# Autodesk Inventor assembly: Robot
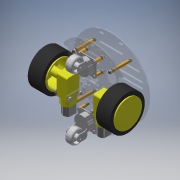
[picture p0: Inventor's stored thumbnail of the model, 180x180]
Saved by Autodesk Inventor 2018 (Build 220112000, 112)
## iProperties
Created: 2018-01-12
Part Number: Robot
Document SubType Name: Assembly
Designer: Kyle
Author: Kyle
## Documents named in this file (12)
- B:\My Documents\Project documentation\Hackathon-2018\Inventor\Robot\Robot.iam
- B:\My Documents\Project documentation\Hackathon-2018\Inventor\Robot\BottomPlate.ipt
- B:\My Documents\Project documentation\Hackathon-2018\Inventor\Robot\MotorMount.ipt
- B:\My Documents\Project documentation\Hackathon-2018\Inventor\Robot\MotorAssembly.iam
- B:\My Documents\Project documentation\Hackathon-2018\Inventor\Robot\MotorScrew.ipt
- B:\My Documents\Project documentation\Hackathon-2018\Inventor\Robot\Nut.ipt
- B:\My Documents\Project documentation\Hackathon-2018\Inventor\Robot\StandoffShort.ipt
- B:\My Documents\Project documentation\Hackathon-2018\Inventor\Robot\Castor.iam
- B:\My Documents\Project documentation\Hackathon-2018\Inventor\Robot\Screw.ipt
- B:\My Documents\Project documentation\Hackathon-2018\Inventor\Robot\StandoffLong.ipt
- B:\My Documents\Project documentation\Hackathon-2018\Inventor\Robot\TopPlate.ipt
- B:\My Documents\Project documentation\Hackathon-2018\Inventor\Robot\WheelAssembly.iam
## Components (52 placed, 11 different names)
1. BottomPlate:1 — Mate:1, Mate:2, Mate:3, Mate:4, Mate:5, Mate:6, Mate:7, Mate:8, Mate:9, Mate:10, Mate:11, Mate:12, Angle:1, Angle:2, Mate:33, Mate:34, Mate:35, Mate:36, Mate:37, Mate:38, Mate:39, Mate:40, Mate:41, Mate:43, Mate:45, Mate:47, Mate:60, Mate:61, Mate:62, Mate:63, Mate:64, Mate:65, Mate:66, Mate:67, Mate:79, Mate:80, Mate:81, Mate:82, Mate:83, Mate:84, Mate:85, Mate:86, Mate:87, Mate:89, Mate:91, Mate:93
2. MotorMount:1 — Mate:1, Mate:2, Mate:3, Mate:14, Mate:29, Mate:31
3. MotorMount:2 — Mate:4, Mate:5, Mate:6, Mate:13, Mate:21, Mate:23
4. MotorMount:3 — Mate:10, Mate:11, Mate:12, Mate:15, Mate:17, Mate:19
5. MotorMount:4 — Mate:7, Mate:8, Mate:9, Mate:16, Mate:25, Mate:27
6. MotorAssembly:1 [sub-assembly] — Mate:13, Angle:1, Mate:14, Mate:22, Mate:24, Mate:109, Mate:110, Mate:111
7. MotorAssembly:2 [sub-assembly] — Mate:15, Angle:2, Mate:16, Mate:18, Mate:20, Mate:106, Mate:107, Mate:108
8. MotorScrew:1 — Mate:17, Mate:18, Mate:26
9. MotorScrew:2 — Mate:19, Mate:20, Mate:28
10. MotorScrew:3 — Mate:23, Mate:24, Mate:30
11. MotorScrew:4 — Mate:21, Mate:22, Mate:32
12. Nut:1 — Mate:29, Mate:30
13. Nut:2 — Mate:31, Mate:32
14. Nut:3 — Mate:27, Mate:28
15. Nut:4 — Mate:25, Mate:26
16. StandoffShort:1 — Mate:36, Mate:40, Mate:42
17. StandoffShort:2 — Mate:35, Mate:37, Mate:48, Mate:50, Mate:51
18. StandoffShort:3 — Mate:34, Mate:39, Mate:44
19. StandoffShort:4 — Mate:33, Mate:38, Mate:46, Mate:49
20. Nut:5 — Mate:47, Mate:48
21. Nut:6 — Mate:45, Mate:46
22. Nut:7 — Mate:41, Mate:42
23. Nut:8 — Mate:43, Mate:44
24. Castor:1 [sub-assembly] — Mate:49, Mate:50, Mate:51, Mate:52, Mate:53, Mate:54, Mate:55, Mate:56, Mate:57, Mate:58, Mate:59
25. Screw:1 — Mate:52, Mate:54
26. Screw:2 — Mate:53, Mate:55
27. Screw:3 — Mate:56, Mate:59
28. Screw:4 — Mate:57, Mate:58
29. Castor:2 [sub-assembly] — Mate:68, Mate:69, Mate:70, Mate:71, Mate:72, Mate:73, Mate:74, Mate:76, Mate:77, Mate:78
30. StandoffShort:5 — Mate:60, Mate:65
31. StandoffShort:6 — Mate:61, Mate:67, Mate:68
32. StandoffShort:7 — Mate:62, Mate:66, Mate:69, Mate:70
33. StandoffShort:8 — Mate:63, Mate:64, Mate:75
34. Screw:5 — Mate:74, Mate:75
35. Screw:6 — Mate:73, Mate:76
36. Screw:7 — Mate:72, Mate:78
37. Screw:8 — Mate:71, Mate:77
38. StandoffLong:1 — Mate:79, Mate:82, Mate:88, Mate:95, Mate:96
39. StandoffLong:2 — Mate:80, Mate:81, Mate:90, Mate:97
40. StandoffLong:3 — Mate:83, Mate:84, Mate:94
41. StandoffLong:4 — Mate:85, Mate:86, Mate:92
42. Nut:9 — Mate:91, Mate:92
43. Nut:10 — Mate:93, Mate:94
44. Nut:11 — Mate:89, Mate:90
45. Nut:12 — Mate:87, Mate:88
46. TopPlate:1 — Mate:95, Mate:96, Mate:97, Mate:98, Mate:99, Mate:100, Mate:101, Mate:102, Mate:103, Mate:104, Mate:105
47. Screw:9 — Mate:98, Mate:99
48. Screw:10 — Mate:102, Mate:103
49. Screw:11 — Mate:100, Mate:101
50. Screw:12 — Mate:104, Mate:105
51. WheelAssembly:1 [sub-assembly] — Mate:106, Mate:107, Mate:108
52. WheelAssembly:2 [sub-assembly] — Mate:109, Mate:110, Mate:111
## Relationships (113: Mate 111, Angle 2)
- Mate:1: BottomPlate:1 ↔ MotorMount:1
- Mate:2: BottomPlate:1 ↔ MotorMount:1
- Mate:3: BottomPlate:1 ↔ MotorMount:1
- Mate:4: BottomPlate:1 ↔ MotorMount:2
- Mate:5: BottomPlate:1 ↔ MotorMount:2
- Mate:6: BottomPlate:1 ↔ MotorMount:2
- Mate:7: BottomPlate:1 ↔ MotorMount:4
- Mate:8: BottomPlate:1 ↔ MotorMount:4
- Mate:9: BottomPlate:1 ↔ MotorMount:4
- Mate:10: BottomPlate:1 ↔ MotorMount:3
- Mate:11: BottomPlate:1 ↔ MotorMount:3
- Mate:12: BottomPlate:1 ↔ MotorMount:3
- Mate:13: MotorMount:2 ↔ MotorAssembly:1
- Angle:1 (0 deg): BottomPlate:1 ↔ MotorAssembly:1
- Mate:14: MotorMount:1 ↔ MotorAssembly:1
- Mate:15: MotorMount:3 ↔ MotorAssembly:2
- Angle:2 (0 deg): BottomPlate:1 ↔ MotorAssembly:2
- Mate:16: MotorMount:4 ↔ MotorAssembly:2
- Mate:17: MotorMount:3 ↔ MotorScrew:1
- Mate:18: MotorAssembly:2 ↔ MotorScrew:1
- Mate:19: MotorMount:3 ↔ MotorScrew:2
- Mate:20: MotorAssembly:2 ↔ MotorScrew:2
- Mate:21: MotorMount:2 ↔ MotorScrew:4
- Mate:22: MotorAssembly:1 ↔ MotorScrew:4
- Mate:23: MotorMount:2 ↔ MotorScrew:3
- Mate:24: MotorAssembly:1 ↔ MotorScrew:3
- Mate:25: MotorMount:4 ↔ Nut:4
- Mate:26: MotorScrew:1 ↔ Nut:4
- Mate:27: MotorMount:4 ↔ Nut:3
- Mate:28: MotorScrew:2 ↔ Nut:3
- Mate:29: MotorMount:1 ↔ Nut:1
- Mate:30: MotorScrew:3 ↔ Nut:1
- Mate:31: MotorMount:1 ↔ Nut:2
- Mate:32: MotorScrew:4 ↔ Nut:2
- Mate:33: BottomPlate:1 ↔ StandoffShort:4
- Mate:34: BottomPlate:1 ↔ StandoffShort:3
- Mate:35: BottomPlate:1 ↔ StandoffShort:2
- Mate:36: BottomPlate:1 ↔ StandoffShort:1
- Mate:37: BottomPlate:1 ↔ StandoffShort:2
- Mate:38: BottomPlate:1 ↔ StandoffShort:4
- Mate:39: BottomPlate:1 ↔ StandoffShort:3
- Mate:40: BottomPlate:1 ↔ StandoffShort:1
- Mate:41: BottomPlate:1 ↔ Nut:7
- Mate:42: StandoffShort:1 ↔ Nut:7
- Mate:43: BottomPlate:1 ↔ Nut:8
- Mate:44: StandoffShort:3 ↔ Nut:8
- Mate:45: BottomPlate:1 ↔ Nut:6
- Mate:46: StandoffShort:4 ↔ Nut:6
- Mate:47: BottomPlate:1 ↔ Nut:5
- Mate:48: StandoffShort:2 ↔ Nut:5
- Mate:49: StandoffShort:4 ↔ Castor:1
- Mate:50: StandoffShort:2 ↔ Castor:1
- Mate:51: StandoffShort:2 ↔ Castor:1
- Mate:52: Castor:1 ↔ Screw:1
- Mate:53: Castor:1 ↔ Screw:2
- Mate:54: Castor:1 ↔ Screw:1
- Mate:55: Castor:1 ↔ Screw:2
- Mate:56: Castor:1 ↔ Screw:3
- Mate:57: Castor:1 ↔ Screw:4
- Mate:58: Castor:1 ↔ Screw:4
- Mate:59: Castor:1 ↔ Screw:3
- Mate:60: BottomPlate:1 ↔ StandoffShort:5
- Mate:61: BottomPlate:1 ↔ StandoffShort:6
- Mate:62: BottomPlate:1 ↔ StandoffShort:7
- Mate:63: BottomPlate:1 ↔ StandoffShort:8
- Mate:64: BottomPlate:1 ↔ StandoffShort:8
- Mate:65: BottomPlate:1 ↔ StandoffShort:5
- Mate:66: BottomPlate:1 ↔ StandoffShort:7
- Mate:67: BottomPlate:1 ↔ StandoffShort:6
- Mate:68: Castor:2 ↔ StandoffShort:6
- Mate:69: Castor:2 ↔ StandoffShort:7
- Mate:70: Castor:2 ↔ StandoffShort:7
- Mate:71: Castor:2 ↔ Screw:8
- Mate:72: Castor:2 ↔ Screw:7
- Mate:73: Castor:2 ↔ Screw:6
- Mate:74: Castor:2 ↔ Screw:5
- Mate:75: StandoffShort:8 ↔ Screw:5
- Mate:76: Castor:2 ↔ Screw:6
- Mate:77: Castor:2 ↔ Screw:8
- Mate:78: Castor:2 ↔ Screw:7
- Mate:79: BottomPlate:1 ↔ StandoffLong:1
- Mate:80: BottomPlate:1 ↔ StandoffLong:2
- Mate:81: BottomPlate:1 ↔ StandoffLong:2
- Mate:82: BottomPlate:1 ↔ StandoffLong:1
- Mate:83: BottomPlate:1 ↔ StandoffLong:3
- Mate:84: BottomPlate:1 ↔ StandoffLong:3
- Mate:85: BottomPlate:1 ↔ StandoffLong:4
- Mate:86: BottomPlate:1 ↔ StandoffLong:4
- Mate:87: BottomPlate:1 ↔ Nut:12
- Mate:88: StandoffLong:1 ↔ Nut:12
- Mate:89: BottomPlate:1 ↔ Nut:11
- Mate:90: StandoffLong:2 ↔ Nut:11
- Mate:91: BottomPlate:1 ↔ Nut:9
- Mate:92: StandoffLong:4 ↔ Nut:9
- Mate:93: BottomPlate:1 ↔ Nut:10
- Mate:94: StandoffLong:3 ↔ Nut:10
- Mate:95: StandoffLong:1 ↔ TopPlate:1
- Mate:96: StandoffLong:1 ↔ TopPlate:1
- Mate:97: StandoffLong:2 ↔ TopPlate:1
- Mate:98: TopPlate:1 ↔ Screw:9
- Mate:99: TopPlate:1 ↔ Screw:9
- Mate:100: TopPlate:1 ↔ Screw:11
- Mate:101: TopPlate:1 ↔ Screw:11
- Mate:102: TopPlate:1 ↔ Screw:10
- Mate:103: TopPlate:1 ↔ Screw:10
- Mate:104: TopPlate:1 ↔ Screw:12
- Mate:105: TopPlate:1 ↔ Screw:12
- Mate:106: MotorAssembly:2 ↔ WheelAssembly:1
- Mate:107: MotorAssembly:2 ↔ WheelAssembly:1
- Mate:108: MotorAssembly:2 ↔ WheelAssembly:1
- Mate:109: MotorAssembly:1 ↔ WheelAssembly:2
- Mate:110: MotorAssembly:1 ↔ WheelAssembly:2
- Mate:111: MotorAssembly:1 ↔ WheelAssembly:2
